# Autodesk Inventor assembly: 75x0y0z_0x0y0z
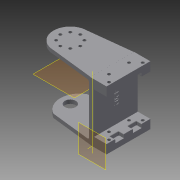
[picture p0: Inventor's stored thumbnail of the model, 180x180]
Saved by Autodesk Inventor 2015 (Build 190159000, 159)
## iProperties
Created: 2016-12-15
Part Number: 75x0y0z_0x0y0z
Document SubType Name: Assembly
Designer: Rudge-Top
Author: Rudge-Top
## Documents named in this file (3)
- C:\Users\Rudge-Top\Documents\RoboticArm\Inventor 2015\Straight Links\75x0y0z_0x0y0z.iam
- C:\Users\Rudge-Top\Documents\RoboticArm\Inventor 2015\Mounts\BaseMount.ipt
- C:\Users\Rudge-Top\Documents\RoboticArm\Inventor 2015\Mounts\Turnmount.ipt
## Components (2 placed, 2 different names)
1. BaseMount:1 — Flush:3, Flush:4, Mate:1
2. Turnmount:1 — Flush:3, Flush:4, Mate:1
## Relationships (3: Flush 2, Mate 1)
- Flush:3: BaseMount:1 ↔ Turnmount:1
- Flush:4: BaseMount:1 ↔ Turnmount:1
- Mate:1: BaseMount:1 ↔ Turnmount:1
